# Autodesk Inventor assembly: arduinoCaseAssembly
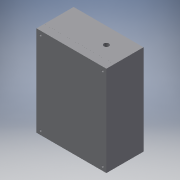
[picture p0: Inventor's stored thumbnail of the model, 180x180]
Saved by Autodesk Inventor 2017 (Build 210142000, 142)
## iProperties
Created: 2017-04-16
Part Number: arduinoCaseAssembly
Document SubType Name: Assembly
Designer: rocke
Author: rocke
## Documents named in this file (3)
- C:\Users\rocke\Documents\Inventor\Eclipse\arduinoCaseAssembly.iam
- C:\Users\rocke\Documents\Inventor\Eclipse\arduinoCase.ipt
- C:\Users\rocke\Documents\Inventor\Eclipse\arduinoCover.ipt
## Components (2 placed, 2 different names)
1. arduinoCase:1 — Mate:1, Flush:1, Flush:2
2. arduinoCover:1 — Mate:1, Flush:1, Flush:2
## Relationships (3: Flush 2, Mate 1)
- Mate:1: arduinoCase:1 ↔ arduinoCover:1
- Flush:1: arduinoCase:1 ↔ arduinoCover:1
- Flush:2: arduinoCase:1 ↔ arduinoCover:1
